# Autodesk Inventor assembly: Structure
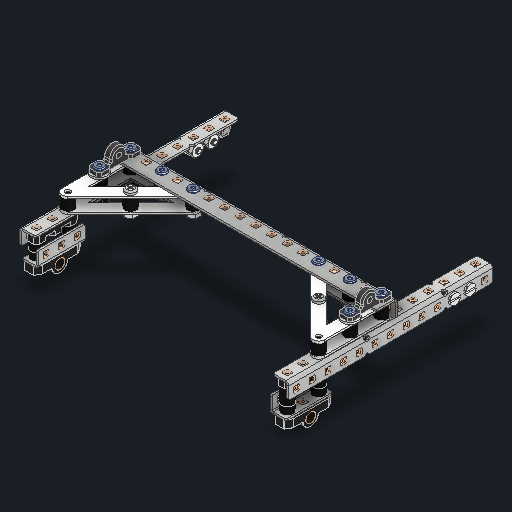
[picture p0: Inventor's stored thumbnail of the model, 512x512]
Saved by Autodesk Inventor 2025.1 (Build 291241000, 241)
## iProperties
Created: 2024-10-21
Part Number: Structure
Document SubType Name: Assembly
Designer: averey
Author: averey
## Documents named in this file (4)
- C:\Users\avere\VEX\High Stakes\CAD\V3\Intake\Floating Stage\Structure.iam
- C:\Users\avere\VEX\High Stakes\CAD\V3\Intake\Floating Stage\Left Angle Structure.iam
- C:\Users\avere\VEX\High Stakes\CAD\V3\Intake\Floating Stage\Right Angle Structure\Right Angle Structure.iam
- C:\Users\avere\VEX\High Stakes\CAD\V3\Intake\Floating Stage\Crossbrace.iam
## Components (3 placed, 3 different names)
1. Left Angle Structure:1 [sub-assembly] — Mate:1, Mate:2, Flush:1, Insert:2, Mate:4
2. Right Angle Structure:1 [sub-assembly] — Flush:2, Mate:3, Flush:3, Insert:3, Mate:5
3. Crossbrace:1 [sub-assembly] — Insert:2, Mate:4, Insert:3, Mate:5
## Relationships (10: Mate 5, Flush 3, Insert 2)
- Mate:1 (96.4184 mm): Left Angle Structure:1
- Mate:2 (-82.55 mm): Left Angle Structure:1
- Flush:1: Left Angle Structure:1
- Flush:2: Right Angle Structure:1
- Mate:3 (-82.55 mm): Right Angle Structure:1
- Flush:3 (96.4184 mm): Right Angle Structure:1
- Insert:2: Left Angle Structure:1 ↔ Crossbrace:1
- Mate:4: Left Angle Structure:1 ↔ Crossbrace:1
- Insert:3: Right Angle Structure:1 ↔ Crossbrace:1
- Mate:5: Right Angle Structure:1 ↔ Crossbrace:1
